# Autodesk Inventor assembly: Intake_Exhaust_Assembly
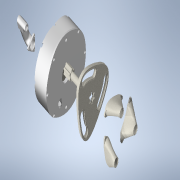
[picture p0: Inventor's stored thumbnail of the model, 180x180]
Saved by Autodesk Inventor 2021 (Build 250183000, 183)
## iProperties
Created: 2021-03-28
Part Number: Intake_Exhaust_Assembly
Document SubType Name: Assembly
Designer: lucia
Author: lucia
## Documents named in this file (10)
- E:\Documents\Inventor\Fixed Rotor Wankel Engine\Assemblies\Intake_Exhaust_Assembly.iam
- E:\Documents\Inventor\Fixed Rotor Wankel Engine\Parts\Rotor_Mount.ipt
- E:\Documents\Inventor\Fixed Rotor Wankel Engine\Parts\Eccentric_Shaft.ipt
- E:\Documents\Inventor\Fixed Rotor Wankel Engine\Parts\Rotor_Geared_6t_Mountable.ipt
- E:\Documents\Inventor\Fixed Rotor Wankel Engine\Parts\Side_Plate_Geared.ipt
- E:\Documents\Inventor\Fixed Rotor Wankel Engine\Parts\Housing.ipt
- E:\Documents\Inventor\Fixed Rotor Wankel Engine\Parts\Side_Plate_Intake_Exhaust.ipt
- E:\Documents\Inventor\Fixed Rotor Wankel Engine\Parts\Exhaust_Plate.ipt
- E:\Documents\Inventor\Fixed Rotor Wankel Engine\Parts\Exhaust Manifold.ipt
- E:\Documents\Inventor\Fixed Rotor Wankel Engine\Parts\Intake Manifold.ipt
## Components (11 placed, 9 different names)
1. Rotor_Mount:1 — Mate:1, Flush:1, Mate:3, Mate:4, Mate:5, Mate:6, Mate:7, Mate:16
2. Eccentric_Shaft:1 — Mate:3, Mate:4, Mate:9, Mate:29
3. Rotor_Geared_6t_Mountable:1 — Mate:5, Mate:6, Mate:7, Mate:8
4. Side_Plate_Geared:1 — Mate:8, Mate:9, Mate:10, Mate:11, Mate:12, Mate:27, Mate:28
5. Housing:1 — Mate:10, Mate:11, Mate:12, Mate:13, Mate:14, Mate:15
6. Side_Plate_Intake_Exhaust:1 — Mate:13, Mate:14, Mate:15, Mate:17
7. Exhaust_Plate:1 — Mate:16, Mate:17, Mate:18, Mate:19, Mate:20, Mate:21, Mate:22, Mate:23, Mate:24, Mate:25, Mate:26
8. Exhaust Manifold:1 — Mate:18, Mate:19, Mate:20
9. Exhaust Manifold:2 — Mate:21, Mate:22, Mate:23
10. Exhaust Manifold:3 — Mate:24, Mate:25, Mate:26
11. Intake Manifold:1 — Mate:27, Mate:28, Mate:29
## Relationships (30: Mate 29, Flush 1)
- Mate:1: Rotor_Mount:1
- Mate:2
- Flush:1: Rotor_Mount:1
- Mate:3: Rotor_Mount:1 ↔ Eccentric_Shaft:1
- Mate:4: Rotor_Mount:1 ↔ Eccentric_Shaft:1
- Mate:5: Rotor_Mount:1 ↔ Rotor_Geared_6t_Mountable:1
- Mate:6: Rotor_Mount:1 ↔ Rotor_Geared_6t_Mountable:1
- Mate:7: Rotor_Mount:1 ↔ Rotor_Geared_6t_Mountable:1
- Mate:8: Rotor_Geared_6t_Mountable:1 ↔ Side_Plate_Geared:1
- Mate:9: Eccentric_Shaft:1 ↔ Side_Plate_Geared:1
- Mate:10: Side_Plate_Geared:1 ↔ Housing:1
- Mate:11: Side_Plate_Geared:1 ↔ Housing:1
- Mate:12: Side_Plate_Geared:1 ↔ Housing:1
- Mate:13: Housing:1 ↔ Side_Plate_Intake_Exhaust:1
- Mate:14: Housing:1 ↔ Side_Plate_Intake_Exhaust:1
- Mate:15: Housing:1 ↔ Side_Plate_Intake_Exhaust:1
- Mate:16: Rotor_Mount:1 ↔ Exhaust_Plate:1
- Mate:17 (152.4 mm): Side_Plate_Intake_Exhaust:1 ↔ Exhaust_Plate:1
- Mate:18 (152.4 mm): Exhaust_Plate:1 ↔ Exhaust Manifold:1
- Mate:19: Exhaust_Plate:1 ↔ Exhaust Manifold:1
- Mate:20: Exhaust_Plate:1 ↔ Exhaust Manifold:1
- Mate:21 (152.4 mm): Exhaust_Plate:1 ↔ Exhaust Manifold:2
- Mate:22: Exhaust_Plate:1 ↔ Exhaust Manifold:2
- Mate:23: Exhaust_Plate:1 ↔ Exhaust Manifold:2
- Mate:24 (152.4 mm): Exhaust_Plate:1 ↔ Exhaust Manifold:3
- Mate:25: Exhaust_Plate:1 ↔ Exhaust Manifold:3
- Mate:26: Exhaust_Plate:1 ↔ Exhaust Manifold:3
- Mate:27 (177.8 mm): Side_Plate_Geared:1 ↔ Intake Manifold:1
- Mate:28: Side_Plate_Geared:1 ↔ Intake Manifold:1
- Mate:29: Eccentric_Shaft:1 ↔ Intake Manifold:1
